# Autodesk Inventor assembly: Elevator Driver
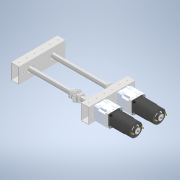
[picture p0: Inventor's stored thumbnail of the model, 180x180]
Saved by Autodesk Inventor 2022 (Build 260153000, 153)
## iProperties
Created: 2021-11-01
Part Number: Elevator Driver
Document SubType Name: Assembly
Designer: merky
Author: merky
## Documents named in this file (7)
- C:\Users\merky\OneDrive\Documents\t3-cad\CAD\2021 Elevator\Elevator Driver.iam
- C:\Users\merky\OneDrive\Documents\t3-cad\CAD\2021 Elevator\Generic Elevator Parts\VersaFrame-Driver.ipt
- C:\Users\merky\OneDrive\Documents\t3-cad\CAD\2021 Elevator\Generic Elevator Parts\Bearing-Thundershaft.ipt
- C:\Users\merky\OneDrive\Documents\t3-cad\CAD\Generic and Stock\VersaPlanetary Single Stage w 775.ipt
- C:\Users\merky\OneDrive\Documents\t3-cad\CAD\2021 Elevator\Generic Elevator Parts\Thundershaft-7.ipt
- C:\Users\merky\OneDrive\Documents\t3-cad\CAD\Generic and Stock\16T 22 Sprocket.ipt
- C:\Users\merky\OneDrive\Documents\t3-cad\CAD\Hex Shaft Collar.ipt
## Components (18 placed, 6 different names)
1. VersaFrame-Driver:1 — Insert:7, Insert:8, Flush:1, Flush:2, Insert:9, Insert:10
2. VersaFrame-Driver:2 — Insert:5, Insert:6, Flush:1, Flush:2, Insert:13
3. Bearing-Thundershaft:5 — Insert:6
4. Bearing-Thundershaft:6 — Insert:5, Insert:11
5. Bearing-Thundershaft:7 — Insert:8
6. Bearing-Thundershaft:8 — Insert:7
7. VersaPlanetary Single Stage w 775:1 — Insert:9
8. VersaPlanetary Single Stage w 775:2 — Insert:10
9. Thundershaft-7:1 — Insert:11, Insert:12, Insert:16, Insert:18, Insert:19, Insert:20
10. 16T 22 Sprocket:1 — Insert:12
11. 16T 22 Sprocket:2 — Insert:14
12. Thundershaft-7:2 — Insert:13, Insert:14, Insert:17, Insert:21
13. 16T 22 Sprocket:4 — Insert:16
14. Hex Shaft Collar:1 — Insert:21
15. Hex Shaft Collar:2 — Insert:17
16. Hex Shaft Collar:3 — Insert:18
17. Hex Shaft Collar:4 — Insert:20
18. Hex Shaft Collar:5 — Insert:19
## Relationships (18: Insert 16, Flush 2)
- Insert:5: VersaFrame-Driver:2 ↔ Bearing-Thundershaft:6
- Insert:6: VersaFrame-Driver:2 ↔ Bearing-Thundershaft:5
- Insert:7: VersaFrame-Driver:1 ↔ Bearing-Thundershaft:8
- Insert:8: VersaFrame-Driver:1 ↔ Bearing-Thundershaft:7
- Flush:1: VersaFrame-Driver:1 ↔ VersaFrame-Driver:2
- Flush:2: VersaFrame-Driver:1 ↔ VersaFrame-Driver:2
- Insert:9 (-40.64 mm): VersaFrame-Driver:1 ↔ VersaPlanetary Single Stage w 775:1
- Insert:10 (-40.64 mm): VersaFrame-Driver:1 ↔ VersaPlanetary Single Stage w 775:2
- Insert:11 (-21.59 mm): Bearing-Thundershaft:6 ↔ Thundershaft-7:1
- Insert:12 (6.35 mm): Thundershaft-7:1 ↔ 16T 22 Sprocket:1
- Insert:13 (-14.224 mm): VersaFrame-Driver:2 ↔ Thundershaft-7:2
- Insert:14 (6.35 mm): 16T 22 Sprocket:2 ↔ Thundershaft-7:2
- Insert:16 (-35.56 mm): Thundershaft-7:1 ↔ 16T 22 Sprocket:4
- Insert:17 (-10.16 mm): Thundershaft-7:2 ↔ Hex Shaft Collar:2
- Insert:18 (-10.16 mm): Thundershaft-7:1 ↔ Hex Shaft Collar:3
- Insert:19 (-25.4 mm): Thundershaft-7:1 ↔ Hex Shaft Collar:5
- Insert:20 (-50.8 mm): Thundershaft-7:1 ↔ Hex Shaft Collar:4
- Insert:21 (-10.16 mm): Thundershaft-7:2 ↔ Hex Shaft Collar:1
